# Autodesk Inventor assembly: inner_frame
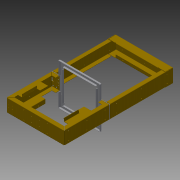
[picture p0: Inventor's stored thumbnail of the model, 180x180]
Saved by Autodesk Inventor 2014 SP2 (Build 180246200, 246)
## iProperties
Created: 2016-05-21
Part Number: inner_frame
Document SubType Name: Assembly
Designer: cruiser
Mass: 557.202 g
Surface Area: 7076.56 cm^2
Volume: 548.411 cm^3
Density: 1.01603 g/cm^3
Author: cruiser
## Documents named in this file (6)
- C:\Users\cruiser\Desktop\models\3d printers\laserresin4\inner_frame.iam
- C:\Users\cruiser\Desktop\models\3d printers\laserresin4\carrier.ipt
- C:\Users\cruiser\Desktop\models\3d printers\laserresin4\frame_inner.ipt
- C:\Users\cruiser\Desktop\models\3d printers\laserresin4\frame_lower.ipt
- C:\Users\cruiser\Desktop\models\3d printers\laserresin4\inner_frame\Design Accelerator\Bolted Connection1.iam
- C:\Users\cruiser\Desktop\models\3d printers\laserresin4\inner_frame\Design Accelerator\Bolted Connection2.iam
## Components (5 placed, 4 different names)
1. carrier:1 — Mate:1, Mate:2, Mate:3, Mate:4, Mate:5, Mate:6, Mate:7, Mate:8
2. frame_inner:1 — Mate:1, Mate:3, Mate:4, Mate:9, Mate:10
3. frame_lower:1 — Mate:2, Mate:5, Mate:6
4. Bolted Connection:1 [sub-assembly] — Mate:7, Mate:8
5. Bolted Connection:2 [sub-assembly] — Mate:9, Mate:10
## Relationships (10: Mate 10)
- Mate:1: carrier:1 ↔ frame_inner:1
- Mate:2: carrier:1 ↔ frame_lower:1
- Mate:3: carrier:1 ↔ frame_inner:1
- Mate:4: carrier:1 ↔ frame_inner:1
- Mate:5: carrier:1 ↔ frame_lower:1
- Mate:6: carrier:1 ↔ frame_lower:1
- Mate:7: carrier:1 ↔ Bolted Connection:1
- Mate:8: carrier:1 ↔ Bolted Connection:1
- Mate:9: frame_inner:1 ↔ Bolted Connection:2
- Mate:10: frame_inner:1 ↔ Bolted Connection:2
